# Autodesk Inventor assembly: Few bended counters
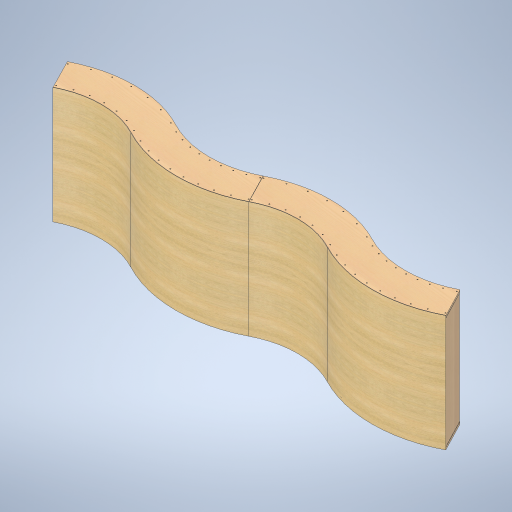
[picture p0: Inventor's stored thumbnail of the model, 512x512]
Saved by Autodesk Inventor 2024 (Build 280153000, 153)
## iProperties
Created: 2021-05-16
Part Number: Few bended counters
Document SubType Name: Assembly
Designer: sauliusd
Author: sauliusd
## Documents named in this file (2)
- C:\W4INV 2024 Design\PROJECTS\Samples\Bended counter\Few bended counters.iam
- C:\W4INV 2024 Design\PROJECTS\Samples\Bended counter\Bended Counter.iam
## Components (2 placed, 1 different names)
1. Bended Counter:1 [sub-assembly] — Mate:1, Flush:1, Flush:2
2. Bended Counter:2 [sub-assembly] — Mate:1, Flush:1, Flush:2
## Relationships (3: Flush 2, Mate 1)
- Mate:1: Bended Counter:1 ↔ Bended Counter:2
- Flush:1: Bended Counter:1 ↔ Bended Counter:2
- Flush:2: Bended Counter:1 ↔ Bended Counter:2
